# Autodesk Inventor assembly: kamerica
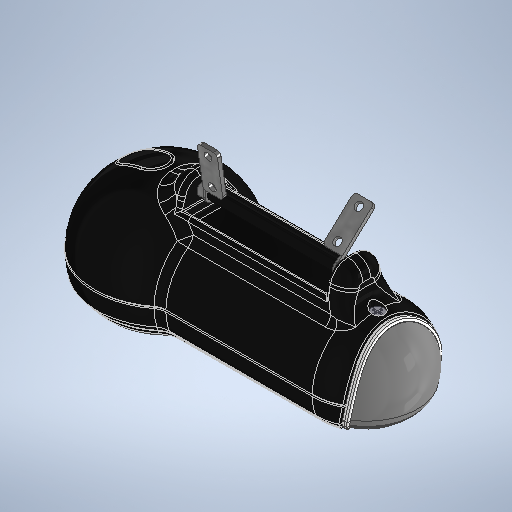
[picture p0: Inventor's stored thumbnail of the model, 512x512]
Saved by Autodesk Inventor 2025.1 (Build 291241020, 241B)
## iProperties
Created: 2011-12-04
Part Number: kamerica
Document SubType Name: Assembly
Designer: 8326d
Sending System: Autodesk Inventor 2012
Preprocessor: Autodesk Inventor 2012
Title: C:\Users\BOZIDAR\Documents\Inventor\quickcam pro 9000\kamerica.stp
Author: BOZIDAR
## Documents named in this file (13)
- C:\Users\8326d\Documents\hobby\CAD\General-Purpose-Robot\camera\kamerica.iam
- C:\Users\8326d\Documents\hobby\CAD\General-Purpose-Robot\camera\kamerica.ipt
- C:\Users\8326d\Documents\hobby\CAD\General-Purpose-Robot\camera\gornji shiny dio.ipt
- C:\Users\8326d\Documents\hobby\CAD\General-Purpose-Robot\camera\objektiv.ipt
- C:\Users\8326d\Documents\hobby\CAD\General-Purpose-Robot\camera\unutrasnja plastika.ipt
- C:\Users\8326d\Documents\hobby\CAD\General-Purpose-Robot\camera\staklence.ipt
- C:\Users\8326d\Documents\hobby\CAD\General-Purpose-Robot\camera\svjetlasce.ipt
- C:\Users\8326d\Documents\hobby\CAD\General-Purpose-Robot\camera\staklo.ipt
- C:\Users\8326d\Documents\hobby\CAD\General-Purpose-Robot\camera\Cross Recessed Flat Countersunk Head Machine Screw - Type I - Metric M2x0,4 x 5.ipt
- C:\Users\8326d\Documents\hobby\CAD\General-Purpose-Robot\camera\majk_Shrinkwrap.ipt
- C:\Users\8326d\Documents\hobby\CAD\General-Purpose-Robot\camera\mrezica.ipt
- C:\Users\8326d\Documents\hobby\CAD\General-Purpose-Robot\camera\hinge.ipt
- C:\Users\8326d\Documents\hobby\CAD\General-Purpose-Robot\camera\hinge-mir.ipt
## Components (12 placed, 12 different names)
1. kamerica_1:1 — 挿入:1, 挿入:2
2. gornji shiny dio_1:1
3. objektiv:1
4. unutrasnja plastika:1
5. staklence:1
6. svjetlasce:1
7. staklo:1
8. Cross Recessed Flat Countersunk Head Machine Screw - Type I - Metric M2x0,4 x 5:1
9. majk_Shrinkwrap:1
10. mrezica:1
11. hinge:1 — 挿入:2
12. hinge-mir:1 — 挿入:1
## Relationships (2: Insert 2)
- 挿入:1 [Insert]: kamerica_1:1 ↔ hinge-mir:1
- 挿入:2 [Insert]: kamerica_1:1 ↔ hinge:1
